# Autodesk Inventor assembly: Funnel Plate Assembly
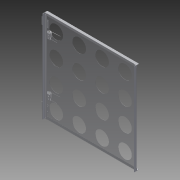
[picture p0: Inventor's stored thumbnail of the model, 180x180]
Saved by Autodesk Inventor 2014 (Build 180170000, 170)
## iProperties
Created: 2014-01-05
Part Number: Funnel Plate Assembly
Document SubType Name: Assembly
Designer: Michael
Author: Michael
## Documents named in this file (6)
- C:\Users\Michael\Documents\Robotics\2014 Season\Funnel Catcher\Funnel Plate Assembly.iam
- C:\Users\Michael\Documents\Robotics\2014 Season\Funnel Catcher\Plastic Funnel PIece.ipt
- C:\Users\Michael\Documents\Robotics\2014 Season\Funnel Catcher\.05 in Aluminum Angle.ipt
- C:\Users\Michael\Documents\Robotics\2014 Season\Funnel Catcher\Flange for Torsion Spring.ipt
- C:\Users\Michael\Documents\Robotics\2014 Season\Funnel Catcher\Door Hinge (1609A120).ipt
- C:\Users\Michael\Documents\Robotics\2014 Season\Funnel Catcher\360 degree Torsion Spring (9271K134).ipt
## Components (13 placed, 5 different names)
1. Plastic Funnel PIece:1 — Insert:23, Insert:24, Insert:25, Insert:26, Insert:39, Insert:40, Insert:41, Insert:42, Insert:43, Insert:44, Insert:45, Insert:46, Insert:47, Insert:48, Insert:49, Insert:50, Angle:1, Angle:2, Insert:51, Insert:52, Insert:53, Insert:54
2. .05 in Aluminum Angle:1 — Insert:25, Insert:26
3. .05 in Aluminum Angle:2 — Insert:23, Insert:24
4. Flange for Torsion Spring:2 — Insert:43, Insert:44
5. Flange for Torsion Spring:4 — Insert:47, Insert:48
6. Flange for Torsion Spring:5 — Mate:2, Insert:45, Insert:46, Mate:4
7. Flange for Torsion Spring:7 — Mate:1, Insert:49, Insert:50, Mate:3
8. Door Hinge (1609A120):1 — Insert:41, Insert:42
9. Door Hinge (1609A120):2 — Insert:39, Insert:40
10. 360 degree Torsion Spring (9271K134):1 — Mate:2, Angle:2, Mate:4
11. 360 degree Torsion Spring (9271K134):2 — Mate:1, Angle:1, Mate:3
12. .05 in Aluminum Angle:3 — Insert:51, Insert:52
13. .05 in Aluminum Angle:4 — Insert:53, Insert:54
## Relationships (26: Insert 20, Mate 4, Angle 2)
- Insert:23: Plastic Funnel PIece:1 ↔ .05 in Aluminum Angle:2
- Insert:24: Plastic Funnel PIece:1 ↔ .05 in Aluminum Angle:2
- Insert:25: Plastic Funnel PIece:1 ↔ .05 in Aluminum Angle:1
- Insert:26: Plastic Funnel PIece:1 ↔ .05 in Aluminum Angle:1
- Insert:39: Plastic Funnel PIece:1 ↔ Door Hinge (1609A120):2
- Insert:40: Plastic Funnel PIece:1 ↔ Door Hinge (1609A120):2
- Insert:41: Plastic Funnel PIece:1 ↔ Door Hinge (1609A120):1
- Insert:42: Plastic Funnel PIece:1 ↔ Door Hinge (1609A120):1
- Mate:1: Flange for Torsion Spring:7 ↔ 360 degree Torsion Spring (9271K134):2
- Mate:2: Flange for Torsion Spring:5 ↔ 360 degree Torsion Spring (9271K134):1
- Insert:43: Plastic Funnel PIece:1 ↔ Flange for Torsion Spring:2
- Insert:44: Plastic Funnel PIece:1 ↔ Flange for Torsion Spring:2
- Insert:45: Plastic Funnel PIece:1 ↔ Flange for Torsion Spring:5
- Insert:46: Plastic Funnel PIece:1 ↔ Flange for Torsion Spring:5
- Insert:47: Plastic Funnel PIece:1 ↔ Flange for Torsion Spring:4
- Insert:48: Plastic Funnel PIece:1 ↔ Flange for Torsion Spring:4
- Insert:49: Plastic Funnel PIece:1 ↔ Flange for Torsion Spring:7
- Insert:50: Plastic Funnel PIece:1 ↔ Flange for Torsion Spring:7
- Angle:1 (90 deg): Plastic Funnel PIece:1 ↔ 360 degree Torsion Spring (9271K134):2
- Angle:2 (90 deg): Plastic Funnel PIece:1 ↔ 360 degree Torsion Spring (9271K134):1
- Mate:3 (4.7625 mm): Flange for Torsion Spring:7 ↔ 360 degree Torsion Spring (9271K134):2
- Mate:4 (4.7625 mm): Flange for Torsion Spring:5 ↔ 360 degree Torsion Spring (9271K134):1
- Insert:51: Plastic Funnel PIece:1 ↔ .05 in Aluminum Angle:3
- Insert:52: Plastic Funnel PIece:1 ↔ .05 in Aluminum Angle:3
- Insert:53: Plastic Funnel PIece:1 ↔ .05 in Aluminum Angle:4
- Insert:54: Plastic Funnel PIece:1 ↔ .05 in Aluminum Angle:4
